# Autodesk Inventor assembly: prueba
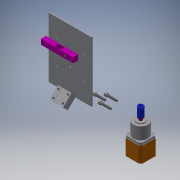
[picture p0: Inventor's stored thumbnail of the model, 180x180]
Saved by Autodesk Inventor 2018 (Build 220112000, 112)
## iProperties
Created: 2019-05-16
Part Number: prueba
Document SubType Name: Assembly
Designer: JLVega003
Author: JLVega003
## Documents named in this file (8)
- C:\Users\JLVega003\Documents\Inventor\Nueva carpeta\Proyecto U\prueba.iam
- C:\Users\JLVega003\Documents\Inventor\Nueva carpeta\Proyecto U\motor con reductora.ipt
- C:\Users\JLVega003\Documents\Inventor\Nueva carpeta\Proyecto U\acople.ipt
- C:\Users\JLVega003\Documents\Inventor\Nueva carpeta\Proyecto U\celda de carga.ipt
- C:\Users\JLVega003\Documents\Inventor\Nueva carpeta\Proyecto U\base superior.ipt
- C:\Users\JLVega003\Documents\Inventor\Content Center Files\R2018\en-US\SS-ISO 4762\ISO 4762 - M5 x 25SS-ISO.ipt
- C:\Users\JLVega003\Documents\Inventor\Content Center Files\R2018\en-US\SS-ISO 4762\ISO 4762 - M5 x 16SS-ISO.ipt
- C:\Users\JLVega003\Documents\Inventor\Nueva carpeta\Proyecto U\cojinete lineal.ipt
## Components (9 placed, 7 different names)
1. motor con reductora:1 — Insert:1
2. acople:1 — Insert:1
3. celda de carga:1 — Insert:2
4. base superior:1 — Insert:2, Insert:3, Angle:1
5. SS ISO 4762 M5 x 16:1 — Insert:3
6. SS ISO 4762 M5 x 25:2
7. SS ISO 4762 M5 x 25:3
8. SS ISO 4762 M5 x 25:4
9. cojinete lineal:1 — Angle:1
## Relationships (4: Insert 3, Angle 1)
- Insert:1 (5 mm): motor con reductora:1 ↔ acople:1
- Insert:2: celda de carga:1 ↔ base superior:1
- Insert:3: base superior:1 ↔ SS ISO 4762 M5 x 16:1
- Angle:1 (45 deg): base superior:1 ↔ cojinete lineal:1
